# Autodesk Inventor assembly: bloc_codeur
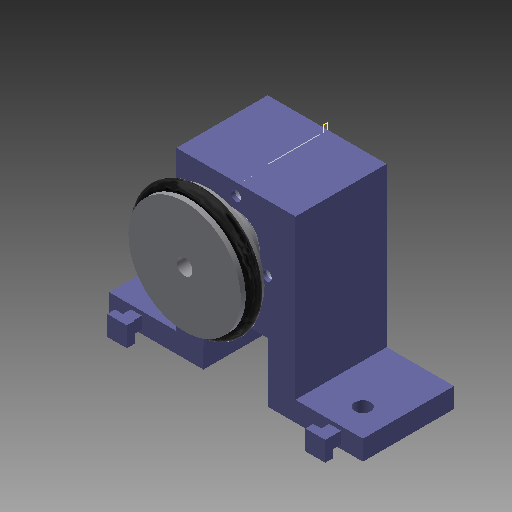
[picture p0: Inventor's stored thumbnail of the model, 512x512]
Saved by Autodesk Inventor 2017 (Build 210142000, 142)
## iProperties
Created: 2017-12-27
Part Number: bloc_codeur
Document SubType Name: Assembly
Designer: franc
Author: franc
## Documents named in this file (4)
- C:\Users\franc\Desktop\EsialRobotik\Mecanique\base_roulante\bloc_codeur.iam
- C:\Users\franc\Desktop\EsialRobotik\Mecanique\base_roulante\composants\codeur_kubler_05.2400_11X2_XXXX.ipt
- C:\Users\franc\Desktop\EsialRobotik\Mecanique\base_roulante\composants\support_codeur.ipt
- C:\Users\franc\Desktop\EsialRobotik\Mecanique\base_roulante\composants\Roue de mesure Scancon 100 mm -ID64.ipt
## Components (3 placed, 3 different names)
1. codeur_kubler_05.2400_11X2_XXXX:1 — Placage:2, Tangente:1, Placage:3, Placage:4, Placage:5
2. support_codeur:1 — Tangente:1, Placage:3, Placage:5
3. Roue de mesure Scancon 100 mm -ID64:1 — Placage:2, Placage:4
## Relationships (5: Mate 4, Tangent 1)
- Placage:2 [Mate]: codeur_kubler_05.2400_11X2_XXXX:1 ↔ Roue de mesure Scancon 100 mm -ID64:1
- Tangente:1: codeur_kubler_05.2400_11X2_XXXX:1 ↔ support_codeur:1
- Placage:3 [Mate]: codeur_kubler_05.2400_11X2_XXXX:1 ↔ support_codeur:1
- Placage:4 [Mate] (1 mm): codeur_kubler_05.2400_11X2_XXXX:1 ↔ Roue de mesure Scancon 100 mm -ID64:1
- Placage:5 [Mate]: codeur_kubler_05.2400_11X2_XXXX:1 ↔ support_codeur:1
